# Autodesk Inventor assembly: 2xiao и компактный короб
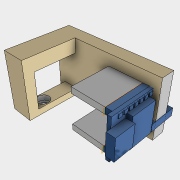
[picture p0: Inventor's stored thumbnail of the model, 180x180]
Saved by Autodesk Inventor 2021.2 (Build 252289000, 289)
## iProperties
Created: 2025-11-19
Part Number: 2xiao и компактный короб
Document SubType Name: Assembly
Designer: Захаров
Author: Захаров
## Documents named in this file (3)
- C:\Users\User\Documents\CaseARHead1\2xiao и компактный короб.iam
- C:\Users\User\Documents\CaseARHead1\ЛЦМК000002.00.00.00.00.06-11 Компактный.ipt
- C:\Users\User\Documents\CaseARHead1\ЛЦМК000002.00.04.00.02.00 2 xiao.iam
## Components (2 placed, 2 different names)
1. ЛЦМК000002.00.00.00.00.06-11 Компактный:1 — Совмещение:1, Совмещение:2, Заподлицо:1
2. ЛЦМК000002.00.04.00.02.00 2 xiao:1 [sub-assembly] — Совмещение:1, Совмещение:2, Заподлицо:1
## Relationships (3: Mate 2, Flush 1)
- Совмещение:1 [Mate]: ЛЦМК000002.00.00.00.00.06-11 Компактный:1 ↔ ЛЦМК000002.00.04.00.02.00 2 xiao:1
- Совмещение:2 [Mate] (3 mm): ЛЦМК000002.00.00.00.00.06-11 Компактный:1 ↔ ЛЦМК000002.00.04.00.02.00 2 xiao:1
- Заподлицо:1 [Flush]: ЛЦМК000002.00.00.00.00.06-11 Компактный:1 ↔ ЛЦМК000002.00.04.00.02.00 2 xiao:1
